# Autodesk Inventor assembly: protector
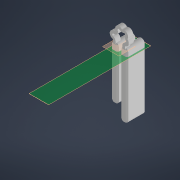
[picture p0: Inventor's stored thumbnail of the model, 180x180]
Saved by Autodesk Inventor 2022 (Build 260153000, 153)
## iProperties
Created: 2023-02-02
Part Number: protector
Document SubType Name: Assembly
Designer: erwin
Author: erwin
## Documents named in this file (5)
- E:\GitHub\ESP32CAMMarauder\parts\protector.iam
- E:\GitHub\ESP32CAMMarauder\parts\pin_header_protector\Part1-01.ipt
- E:\GitHub\ESP32CAMMarauder\parts\pin_header_protector.ipt
- E:\GitHub\ESP32CAMMarauder\parts\pin_header_protector\pin_header_protector-02.ipt
- E:\GitHub\ESP32CAMMarauder\parts\string2.ipt
## Components (3 placed, 3 different names)
1. Part1-01:1 — Mate:1, Flush:1, Tangent:1
2. pin_header_protector-02:2 — Mate:1, Flush:1, Tangent:2, Flush:2
3. string2:1 — Flush:2
## Relationships (8: Mate 2, Flush 2, Angle 2, Tangent 2)
- Mate:1 (1 mm): Part1-01:1 ↔ pin_header_protector-02:2
- Flush:1: Part1-01:1 ↔ pin_header_protector-02:2
- Angle:1 (0 deg)
- Tangent:1: Part1-01:1
- Angle:2 (0 deg)
- Tangent:2: pin_header_protector-02:2
- Mate:2
- Flush:2: pin_header_protector-02:2 ↔ string2:1
